# Autodesk Inventor assembly: repeated section(4)
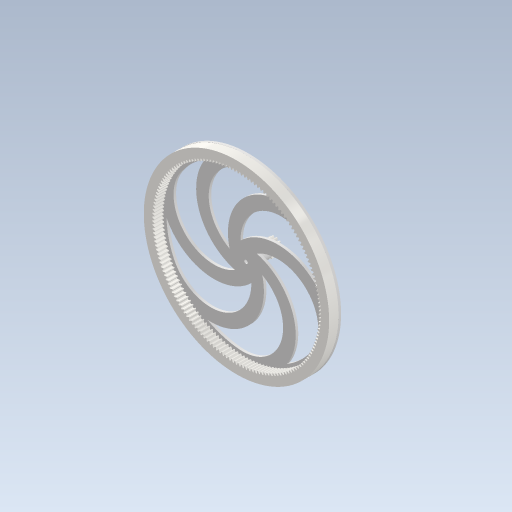
[picture p0: Inventor's stored thumbnail of the model, 512x512]
Saved by Autodesk Inventor 2023 (Build 270158000, 158)
## iProperties
Created: 2023-03-30
Part Number: repeated section(4)
Document SubType Name: Assembly
Designer: dverd
Author: dverd
## Documents named in this file (4)
- C:\Users\dverd\OneDrive\Documents\ME\ME 354\turbine lab 2.0\CAD\repeated section(4).iam
- C:\Users\dverd\OneDrive\Documents\ME\ME 354\turbine lab 2.0\CAD\internal gear.ipt
- C:\Users\dverd\OneDrive\Documents\ME\ME 354\turbine lab 2.0\CAD\gear backing.ipt
- C:\Users\dverd\OneDrive\Documents\ME\ME 354\turbine lab 2.0\CAD\small gear.ipt
## Components (3 placed, 3 different names)
1. Spur Gear2:1 — Mate:1, Mate:2
2. gear backing:1 — Mate:1, Mate:2, Mate:3, Mate:4
3. Spur Gear1:1 — Mate:3, Mate:4
## Relationships (4: Mate 4)
- Mate:1: Spur Gear2:1 ↔ gear backing:1
- Mate:2: Spur Gear2:1 ↔ gear backing:1
- Mate:3: gear backing:1 ↔ Spur Gear1:1
- Mate:4: gear backing:1 ↔ Spur Gear1:1
